# Autodesk Inventor assembly: Battery_pack
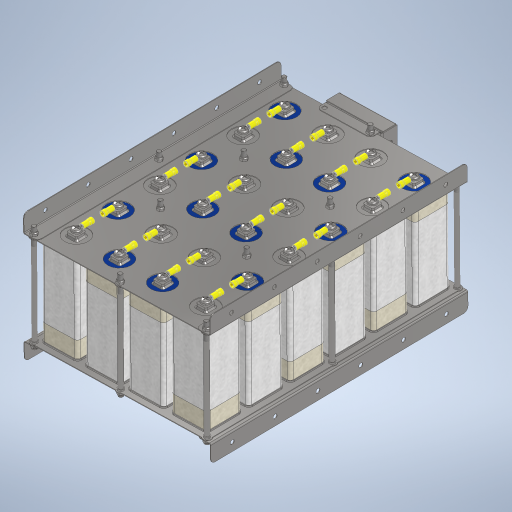
[picture p0: Inventor's stored thumbnail of the model, 512x512]
Saved by Autodesk Inventor 2023 (Build 270158000, 158)
## iProperties
Created: 2022-09-24
Part Number: Battery_pack
Document SubType Name: Assembly
Designer: dms01
Author: dms01
## Documents named in this file (16)
- D:\NEXT SPACE Lab\NaS battery\FINAL PROJECT\Battery_pack.iam
- D:\NEXT SPACE Lab\NaS battery\Frame.ipt
- D:\NEXT SPACE Lab\NaS battery\Square_cell.iam
- C:\Users\dms01\Documents\Inventor\Content Center Files\R2023\ru-RU\Stud GOST 22036-76\Шпилька M6-6g×140 ГОСТ 22036-76.ipt
- C:\Users\dms01\Documents\Inventor\Content Center Files\R2023\ru-RU\ANSI B18.16.3M(2)\ANSI B18.16.3M - Property Class 5 and 10 - Metric M5 x 0.8 Металлич..ipt
- C:\Users\dms01\Documents\Inventor\Content Center Files\R2023\ru-RU\Terminal Ring\#14 Terminal Ring 12 - 10 AWG.ipt
- C:\Users\dms01\Documents\Inventor\Content Center Files\R2023\ru-RU\KS B 1023  H (2)\KS B 1023 - A  M 6 x 8 - H(1).ipt
- C:\Users\dms01\Documents\Inventor\Content Center Files\R2023\ru-RU\D-Sub Female Crimp\D-Sub Female Crimp 9CKT.ipt
- D:\NEXT SPACE Lab\NaS battery\PCB_cover.ipt
- C:\Users\dms01\Documents\Inventor\Content Center Files\R2023\ru-RU\KS B 1023  H (2)\KS B 1023 - A  M 3 x 4 - H(1).ipt
- D:\NEXT SPACE Lab\NaS battery\Side_bar.ipt
- D:\NEXT SPACE Lab\NaS battery\Battery_pack\AIP\FEA\e3tpfgf5s.fins
- D:\NEXT SPACE Lab\NaS battery\Battery_pack\AIP\FEA\e3tpfgf6o.fsat
- D:\NEXT SPACE Lab\NaS battery\Battery_pack\AIP\FEA\e3tpfgf6o.ftes
- D:\NEXT SPACE Lab\NaS battery\Battery_pack\AIP\FEA\e3tpfgf6o.fwiz
- D:\NEXT SPACE Lab\NaS battery\Battery_pack\AIP\FEA\e3tpfghts.fmsh
## Components (168 placed, 10 different names)
1. Frame:1 — Жесткий:4, Вставка:1, Вставка:2, Вставка:3, Вставка:4, Вставка:5, Вставка:6, Вставка:7, Вставка:8, Вставка:9, Вставка:10, Вставка:11, Вставка:12, Вставка:14, Вставка:15, Вставка:16, Вставка:17, Вставка:19, Вставка:23, Жесткий:6, Жесткий:7, Жесткий:8, Жесткий:9, Жесткий:10, Жесткий:11, Жесткий:12, Жесткий:13, Жесткий:14, Жесткий:15, Жесткий:16, Симметрия:1, Жесткий:18, Жесткий:20, Жесткий:22, Жесткий:24, Жесткий:26, Жесткий:28, С поворотом:54, С поворотом:55
2. Frame:2 — Жесткий:5, Вставка:26, Вставка:28, Вставка:29, Вставка:30, Вставка:32, Симметрия:1, Жесткий:17, Жесткий:19, Жесткий:21, Жесткий:23, Жесткий:25, Жесткий:27, С поворотом:53, С поворотом:56, С поворотом:57
3. PCB_cover:1 — С поворотом:46, С поворотом:53, Вставка:104
4. D-Sub розетка, контакты под обжим D-Sub Female Crimp 9CKT:1 — С поворотом:46, Вставка:85, Вставка:86
5. Side_bar:1 — С поворотом:57, Вставка:92, Вставка:93, Вставка:94
6. Side_bar:2 — С поворотом:54, Вставка:101, Вставка:102, Вставка:103
7. Side_bar:3 — С поворотом:56, Вставка:95, Вставка:96, Вставка:97
8. Side_bar:4 — С поворотом:55, Вставка:98, Вставка:99, Вставка:100
9. Шпилька ГОСТ 22036-76 M6-6g×140:1 — Вставка:1
10. Шпилька ГОСТ 22036-76 M6-6g×140:2 — Вставка:2
11. Шпилька ГОСТ 22036-76 M6-6g×140:3 — Вставка:3
12. Шпилька ГОСТ 22036-76 M6-6g×140:4 — Вставка:4
13. Шпилька ГОСТ 22036-76 M6-6g×140:5 — Вставка:5
14. Шпилька ГОСТ 22036-76 M6-6g×140:6 — Вставка:6
15. Шпилька ГОСТ 22036-76 M6-6g×140:7 — Вставка:7
16. Шпилька ГОСТ 22036-76 M6-6g×140:8 — Вставка:8
17. Шпилька ГОСТ 22036-76 M6-6g×140:9 — Вставка:9
18. Шпилька ГОСТ 22036-76 M6-6g×140:10 — Вставка:10
19. Шпилька ГОСТ 22036-76 M6-6g×140:11 — Вставка:11
20. Шпилька ГОСТ 22036-76 M6-6g×140:12 — Вставка:12
21. Гайка шестигранная самоконтрящаяся - Сталь метрическая Property Class 5 and 10 - Metric M5 x 0.8 Металлич.:21 — Вставка:92
22. Гайка шестигранная самоконтрящаяся - Сталь метрическая Property Class 5 and 10 - Metric M5 x 0.8 Металлич.:22 — Вставка:93
23. Гайка шестигранная самоконтрящаяся - Сталь метрическая Property Class 5 and 10 - Metric M5 x 0.8 Металлич.:23 — Вставка:94
24. Гайка шестигранная самоконтрящаяся - Сталь метрическая Property Class 5 and 10 - Metric M5 x 0.8 Металлич.:24 — Вставка:95
25. Гайка шестигранная самоконтрящаяся - Сталь метрическая Property Class 5 and 10 - Metric M5 x 0.8 Металлич.:25 — Вставка:96
26. Гайка шестигранная самоконтрящаяся - Сталь метрическая Property Class 5 and 10 - Metric M5 x 0.8 Металлич.:26 — Вставка:97
27. Гайка шестигранная самоконтрящаяся - Сталь метрическая Property Class 5 and 10 - Metric M5 x 0.8 Металлич.:27 — Вставка:98
28. Гайка шестигранная самоконтрящаяся - Сталь метрическая Property Class 5 and 10 - Metric M5 x 0.8 Металлич.:28 — Вставка:99
29. Гайка шестигранная самоконтрящаяся - Сталь метрическая Property Class 5 and 10 - Metric M5 x 0.8 Металлич.:29 — Вставка:100
30. Гайка шестигранная самоконтрящаяся - Сталь метрическая Property Class 5 and 10 - Metric M5 x 0.8 Металлич.:30 — Вставка:101
31. Гайка шестигранная самоконтрящаяся - Сталь метрическая Property Class 5 and 10 - Metric M5 x 0.8 Металлич.:31 — Вставка:102
32. Гайка шестигранная самоконтрящаяся - Сталь метрическая Property Class 5 and 10 - Metric M5 x 0.8 Металлич.:32 — Вставка:103
33. Гайка шестигранная самоконтрящаяся - Сталь метрическая Property Class 5 and 10 - Metric M5 x 0.8 Металлич.:33 — Вставка:104
34. Гайка шестигранная самоконтрящаяся - Сталь метрическая Property Class 5 and 10 - Metric M5 x 0.8 Металлич.:2 — Вставка:14
35. Гайка шестигранная самоконтрящаяся - Сталь метрическая Property Class 5 and 10 - Metric M5 x 0.8 Металлич.:3 — Вставка:15
36. Гайка шестигранная самоконтрящаяся - Сталь метрическая Property Class 5 and 10 - Metric M5 x 0.8 Металлич.:4 — Вставка:16
37. Гайка шестигранная самоконтрящаяся - Сталь метрическая Property Class 5 and 10 - Metric M5 x 0.8 Металлич.:5 — Вставка:17
38. Гайка шестигранная самоконтрящаяся - Сталь метрическая Property Class 5 and 10 - Metric M5 x 0.8 Металлич.:7 — Вставка:19
39. Гайка шестигранная самоконтрящаяся - Сталь метрическая Property Class 5 and 10 - Metric M5 x 0.8 Металлич.:11 — Вставка:23
40. Гайка шестигранная самоконтрящаяся - Сталь метрическая Property Class 5 and 10 - Metric M5 x 0.8 Металлич.:14 — Вставка:26
41. Гайка шестигранная самоконтрящаяся - Сталь метрическая Property Class 5 and 10 - Metric M5 x 0.8 Металлич.:16 — Вставка:28
42. Гайка шестигранная самоконтрящаяся - Сталь метрическая Property Class 5 and 10 - Metric M5 x 0.8 Металлич.:17 — Вставка:29
43. Гайка шестигранная самоконтрящаяся - Сталь метрическая Property Class 5 and 10 - Metric M5 x 0.8 Металлич.:18 — Вставка:30
44. Гайка шестигранная самоконтрящаяся - Сталь метрическая Property Class 5 and 10 - Metric M5 x 0.8 Металлич.:20 — Вставка:32
45. Square_cell:8 [sub-assembly] — Жесткий:4, Жесткий:5, С поворотом:1, С поворотом:50
46. Square_cell:13 [sub-assembly] — Жесткий:10, С поворотом:10, С поворотом:11
47. Square_cell:12 [sub-assembly] — Жесткий:9, С поворотом:8, С поворотом:9
48. Square_cell:11 [sub-assembly] — Жесткий:8, С поворотом:6, С поворотом:7
49. Square_cell:10 [sub-assembly] — Жесткий:7, С поворотом:4, С поворотом:5
50. Square_cell:9 [sub-assembly] — Жесткий:6, С поворотом:2, С поворотом:3
51. Square_cell:19 [sub-assembly] — Жесткий:16, С поворотом:22, С поворотом:48
52. Square_cell:18 [sub-assembly] — Жесткий:15, С поворотом:20, С поворотом:21
53. Square_cell:17 [sub-assembly] — Жесткий:14, С поворотом:18, С поворотом:19
54. Square_cell:16 [sub-assembly] — Жесткий:13, С поворотом:16, С поворотом:17
55. Square_cell:15 [sub-assembly] — Жесткий:12, С поворотом:14, С поворотом:15
56. Square_cell:14 [sub-assembly] — Жесткий:11, С поворотом:12, С поворотом:13
57. Square_cell:20 [sub-assembly] — Жесткий:17, С поворотом:32, С поворотом:33
58. Square_cell:21 [sub-assembly] — Жесткий:18, С поворотом:30, С поворотом:31
59. Square_cell:22 [sub-assembly] — Жесткий:19, С поворотом:25, С поворотом:29
60. Square_cell:23 [sub-assembly] — Жесткий:20, С поворотом:26, С поворотом:28
61. Square_cell:24 [sub-assembly] — Жесткий:21, С поворотом:24, С поворотом:27
62. Square_cell:25 [sub-assembly] — Жесткий:22, С поворотом:23, С поворотом:47
63. Square_cell:26 [sub-assembly] — Жесткий:23, С поворотом:44, С поворотом:51
64. Square_cell:27 [sub-assembly] — Жесткий:24, С поворотом:40, С поворотом:43
65. Square_cell:28 [sub-assembly] — Жесткий:25, С поворотом:39, С поворотом:42
66. Square_cell:29 [sub-assembly] — Жесткий:26, С поворотом:38, С поворотом:41
67. Square_cell:30 [sub-assembly] — Жесткий:27, С поворотом:36, С поворотом:37
68. Square_cell:31 [sub-assembly] — Жесткий:28, С поворотом:34, С поворотом:35
69. Кольцевой зажим #14 Terminal Ring 12 - 10 AWG:45 — С поворотом:47, Вставка:89
70. Кольцевой зажим #14 Terminal Ring 12 - 10 AWG:46 — С поворотом:48, С поворотом:49
71. Кольцевой зажим #14 Terminal Ring 12 - 10 AWG:47 — С поворотом:49, Вставка:90
72. Кольцевой зажим #14 Terminal Ring 12 - 10 AWG:48 — С поворотом:50, С поворотом:52
73. Кольцевой зажим #14 Terminal Ring 12 - 10 AWG:49 — С поворотом:51, Вставка:88
74. Кольцевой зажим #14 Terminal Ring 12 - 10 AWG:50 — С поворотом:52, Вставка:91
75. Кольцевой зажим #14 Terminal Ring 12 - 10 AWG:1 — С поворотом:1, Вставка:57
76. Кольцевой зажим #14 Terminal Ring 12 - 10 AWG:2 — С поворотом:2, Вставка:56
77. Кольцевой зажим #14 Terminal Ring 12 - 10 AWG:3 — С поворотом:10, Вставка:48
78. Кольцевой зажим #14 Terminal Ring 12 - 10 AWG:4 — С поворотом:9, Вставка:46
79. Кольцевой зажим #14 Terminal Ring 12 - 10 AWG:5 — С поворотом:7, Вставка:69
80. Кольцевой зажим #14 Terminal Ring 12 - 10 AWG:6 — С поворотом:8, Вставка:68
81. Кольцевой зажим #14 Terminal Ring 12 - 10 AWG:7 — С поворотом:5, Вставка:49
82. Кольцевой зажим #14 Terminal Ring 12 - 10 AWG:8 — С поворотом:6, Вставка:47
83. Кольцевой зажим #14 Terminal Ring 12 - 10 AWG:9 — С поворотом:3, Вставка:80
84. Кольцевой зажим #14 Terminal Ring 12 - 10 AWG:10 — С поворотом:4, Вставка:73
85. Кольцевой зажим #14 Terminal Ring 12 - 10 AWG:11 — С поворотом:20, Вставка:79
86. Кольцевой зажим #14 Terminal Ring 12 - 10 AWG:12 — С поворотом:19, Вставка:74
87. Кольцевой зажим #14 Terminal Ring 12 - 10 AWG:13 — С поворотом:18, Вставка:50
88. Кольцевой зажим #14 Terminal Ring 12 - 10 AWG:14 — С поворотом:17, Вставка:45
89. Кольцевой зажим #14 Terminal Ring 12 - 10 AWG:15 — С поворотом:16, Вставка:70
90. Кольцевой зажим #14 Terminal Ring 12 - 10 AWG:16 — С поворотом:15, Вставка:67
91. Кольцевой зажим #14 Terminal Ring 12 - 10 AWG:17 — С поворотом:14, Вставка:42
92. Кольцевой зажим #14 Terminal Ring 12 - 10 AWG:18 — С поворотом:13, Вставка:39
93. Кольцевой зажим #14 Terminal Ring 12 - 10 AWG:19 — С поворотом:12, Вставка:62
94. Кольцевой зажим #14 Terminal Ring 12 - 10 AWG:20 — С поворотом:11, Вставка:61
95. Кольцевой зажим #14 Terminal Ring 12 - 10 AWG:21 — С поворотом:22, Вставка:58
96. Кольцевой зажим #14 Terminal Ring 12 - 10 AWG:22 — С поворотом:21, Вставка:55
97. Кольцевой зажим #14 Terminal Ring 12 - 10 AWG:23 — С поворотом:23, Вставка:59
98. Кольцевой зажим #14 Terminal Ring 12 - 10 AWG:24 — С поворотом:25, Вставка:43
99. Кольцевой зажим #14 Terminal Ring 12 - 10 AWG:25 — С поворотом:27, Вставка:78
100. Кольцевой зажим #14 Terminal Ring 12 - 10 AWG:26 — С поворотом:29, Вставка:71
101. Кольцевой зажим #14 Terminal Ring 12 - 10 AWG:27 — С поворотом:40, Вставка:77
102. Кольцевой зажим #14 Terminal Ring 12 - 10 AWG:28 — С поворотом:38, Вставка:72
103. Кольцевой зажим #14 Terminal Ring 12 - 10 AWG:29 — С поворотом:37, Вставка:65
104. Кольцевой зажим #14 Terminal Ring 12 - 10 AWG:30 — С поворотом:35, Вставка:37
105. Кольцевой зажим #14 Terminal Ring 12 - 10 AWG:31 — С поворотом:33, Вставка:63
106. Кольцевой зажим #14 Terminal Ring 12 - 10 AWG:32 — С поворотом:32, Вставка:38
107. Кольцевой зажим #14 Terminal Ring 12 - 10 AWG:33 — С поворотом:31, Вставка:40
108. Кольцевой зажим #14 Terminal Ring 12 - 10 AWG:34 — С поворотом:34, Вставка:64
109. Кольцевой зажим #14 Terminal Ring 12 - 10 AWG:35 — С поворотом:36, Вставка:41
110. Кольцевой зажим #14 Terminal Ring 12 - 10 AWG:36 — С поворотом:39, Вставка:76
111. Кольцевой зажим #14 Terminal Ring 12 - 10 AWG:37 — С поворотом:41, Вставка:44
112. Кольцевой зажим #14 Terminal Ring 12 - 10 AWG:38 — С поворотом:42, Вставка:52
113. Кольцевой зажим #14 Terminal Ring 12 - 10 AWG:39 — С поворотом:30, Вставка:66
114. Кольцевой зажим #14 Terminal Ring 12 - 10 AWG:40 — С поворотом:28, Вставка:75
115. Кольцевой зажим #14 Terminal Ring 12 - 10 AWG:41 — С поворотом:26, Вставка:51
116. Кольцевой зажим #14 Terminal Ring 12 - 10 AWG:42 — С поворотом:24, Вставка:54
117. Кольцевой зажим #14 Terminal Ring 12 - 10 AWG:43 — С поворотом:43, Вставка:53
118. Кольцевой зажим #14 Terminal Ring 12 - 10 AWG:44 — С поворотом:44, Вставка:60
119. KS B 1023 H - метрическая A  M 6 x 8 - H:45 — Вставка:88
120. KS B 1023 H - метрическая A  M 6 x 8 - H:46 — Вставка:89
121. KS B 1023 H - метрическая A  M 6 x 8 - H:47 — Вставка:90
122. KS B 1023 H - метрическая A  M 6 x 8 - H:48 — Вставка:91
123. KS B 1023 H - метрическая A  M 3 x 4 - H:1 — Вставка:85
124. KS B 1023 H - метрическая A  M 3 x 4 - H:2 — Вставка:86
125. KS B 1023 H - метрическая A  M 6 x 8 - H:1 — Вставка:37
126. KS B 1023 H - метрическая A  M 6 x 8 - H:2 — Вставка:38
127. KS B 1023 H - метрическая A  M 6 x 8 - H:3 — Вставка:39
128. KS B 1023 H - метрическая A  M 6 x 8 - H:4 — Вставка:40
129. KS B 1023 H - метрическая A  M 6 x 8 - H:5 — Вставка:41
130. KS B 1023 H - метрическая A  M 6 x 8 - H:6 — Вставка:42
131. KS B 1023 H - метрическая A  M 6 x 8 - H:7 — Вставка:43
132. KS B 1023 H - метрическая A  M 6 x 8 - H:8 — Вставка:44
133. KS B 1023 H - метрическая A  M 6 x 8 - H:9 — Вставка:45
134. KS B 1023 H - метрическая A  M 6 x 8 - H:10 — Вставка:46
135. KS B 1023 H - метрическая A  M 6 x 8 - H:11 — Вставка:47
136. KS B 1023 H - метрическая A  M 6 x 8 - H:12 — Вставка:48
137. KS B 1023 H - метрическая A  M 6 x 8 - H:13 — Вставка:49
138. KS B 1023 H - метрическая A  M 6 x 8 - H:14 — Вставка:50
139. KS B 1023 H - метрическая A  M 6 x 8 - H:15 — Вставка:51
140. KS B 1023 H - метрическая A  M 6 x 8 - H:16 — Вставка:52
141. KS B 1023 H - метрическая A  M 6 x 8 - H:17 — Вставка:53
142. KS B 1023 H - метрическая A  M 6 x 8 - H:18 — Вставка:54
143. KS B 1023 H - метрическая A  M 6 x 8 - H:19 — Вставка:55
144. KS B 1023 H - метрическая A  M 6 x 8 - H:20 — Вставка:56
145. KS B 1023 H - метрическая A  M 6 x 8 - H:21 — Вставка:57
146. KS B 1023 H - метрическая A  M 6 x 8 - H:22 — Вставка:58
147. KS B 1023 H - метрическая A  M 6 x 8 - H:23 — Вставка:59
148. KS B 1023 H - метрическая A  M 6 x 8 - H:24 — Вставка:60
149. KS B 1023 H - метрическая A  M 6 x 8 - H:25 — Вставка:61
150. KS B 1023 H - метрическая A  M 6 x 8 - H:26 — Вставка:62
151. KS B 1023 H - метрическая A  M 6 x 8 - H:27 — Вставка:63
152. KS B 1023 H - метрическая A  M 6 x 8 - H:28 — Вставка:64
153. KS B 1023 H - метрическая A  M 6 x 8 - H:29 — Вставка:65
154. KS B 1023 H - метрическая A  M 6 x 8 - H:30 — Вставка:66
155. KS B 1023 H - метрическая A  M 6 x 8 - H:31 — Вставка:67
156. KS B 1023 H - метрическая A  M 6 x 8 - H:32 — Вставка:68
157. KS B 1023 H - метрическая A  M 6 x 8 - H:33 — Вставка:69
158. KS B 1023 H - метрическая A  M 6 x 8 - H:34 — Вставка:70
159. KS B 1023 H - метрическая A  M 6 x 8 - H:35 — Вставка:71
160. KS B 1023 H - метрическая A  M 6 x 8 - H:36 — Вставка:72
161. KS B 1023 H - метрическая A  M 6 x 8 - H:37 — Вставка:73
162. KS B 1023 H - метрическая A  M 6 x 8 - H:38 — Вставка:74
163. KS B 1023 H - метрическая A  M 6 x 8 - H:39 — Вставка:75
164. KS B 1023 H - метрическая A  M 6 x 8 - H:40 — Вставка:76
165. KS B 1023 H - метрическая A  M 6 x 8 - H:41 — Вставка:77
166. KS B 1023 H - метрическая A  M 6 x 8 - H:42 — Вставка:78
167. KS B 1023 H - метрическая A  M 6 x 8 - H:43 — Вставка:79
168. KS B 1023 H - метрическая A  M 6 x 8 - H:44 — Вставка:80
## Relationships (168: Insert 86, RevoluteJoint 56, WeldJoint 25, Symmetry 1)
- Жесткий:4 [WeldJoint]: Frame:1 ↔ Square_cell:8
- Жесткий:5 [WeldJoint]: Frame:2 ↔ Square_cell:8
- Вставка:1 [Insert]: Frame:1 ↔ Шпилька ГОСТ 22036-76 M6-6g×140:1
- Вставка:2 [Insert]: Frame:1 ↔ Шпилька ГОСТ 22036-76 M6-6g×140:2
- Вставка:3 [Insert]: Frame:1 ↔ Шпилька ГОСТ 22036-76 M6-6g×140:3
- Вставка:4 [Insert]: Frame:1 ↔ Шпилька ГОСТ 22036-76 M6-6g×140:4
- Вставка:5 [Insert]: Frame:1 ↔ Шпилька ГОСТ 22036-76 M6-6g×140:5
- Вставка:6 [Insert]: Frame:1 ↔ Шпилька ГОСТ 22036-76 M6-6g×140:6
- Вставка:7 [Insert]: Frame:1 ↔ Шпилька ГОСТ 22036-76 M6-6g×140:7
- Вставка:8 [Insert]: Frame:1 ↔ Шпилька ГОСТ 22036-76 M6-6g×140:8
- Вставка:9 [Insert]: Frame:1 ↔ Шпилька ГОСТ 22036-76 M6-6g×140:9
- Вставка:10 [Insert]: Frame:1 ↔ Шпилька ГОСТ 22036-76 M6-6g×140:10
- Вставка:11 [Insert]: Frame:1 ↔ Шпилька ГОСТ 22036-76 M6-6g×140:11
- Вставка:12 [Insert]: Frame:1 ↔ Шпилька ГОСТ 22036-76 M6-6g×140:12
- Вставка:14 [Insert]: Frame:1 ↔ Гайка шестигранная самоконтрящаяся - Сталь метрическая Property Class 5 and 10 - Metric M5 x 0.8 Металлич.:2
- Вставка:15 [Insert]: Frame:1 ↔ Гайка шестигранная самоконтрящаяся - Сталь метрическая Property Class 5 and 10 - Metric M5 x 0.8 Металлич.:3
- Вставка:16 [Insert]: Frame:1 ↔ Гайка шестигранная самоконтрящаяся - Сталь метрическая Property Class 5 and 10 - Metric M5 x 0.8 Металлич.:4
- Вставка:17 [Insert]: Frame:1 ↔ Гайка шестигранная самоконтрящаяся - Сталь метрическая Property Class 5 and 10 - Metric M5 x 0.8 Металлич.:5
- Вставка:19 [Insert]: Frame:1 ↔ Гайка шестигранная самоконтрящаяся - Сталь метрическая Property Class 5 and 10 - Metric M5 x 0.8 Металлич.:7
- Вставка:23 [Insert]: Frame:1 ↔ Гайка шестигранная самоконтрящаяся - Сталь метрическая Property Class 5 and 10 - Metric M5 x 0.8 Металлич.:11
- Вставка:26 [Insert]: Frame:2 ↔ Гайка шестигранная самоконтрящаяся - Сталь метрическая Property Class 5 and 10 - Metric M5 x 0.8 Металлич.:14
- Вставка:28 [Insert]: Frame:2 ↔ Гайка шестигранная самоконтрящаяся - Сталь метрическая Property Class 5 and 10 - Metric M5 x 0.8 Металлич.:16
- Вставка:29 [Insert]: Frame:2 ↔ Гайка шестигранная самоконтрящаяся - Сталь метрическая Property Class 5 and 10 - Metric M5 x 0.8 Металлич.:17
- Вставка:30 [Insert]: Frame:2 ↔ Гайка шестигранная самоконтрящаяся - Сталь метрическая Property Class 5 and 10 - Metric M5 x 0.8 Металлич.:18
- Вставка:32 [Insert]: Frame:2 ↔ Гайка шестигранная самоконтрящаяся - Сталь метрическая Property Class 5 and 10 - Metric M5 x 0.8 Металлич.:20
- Жесткий:6 [WeldJoint]: Frame:1 ↔ Square_cell:9
- Жесткий:7 [WeldJoint]: Frame:1 ↔ Square_cell:10
- Жесткий:8 [WeldJoint]: Frame:1 ↔ Square_cell:11
- Жесткий:9 [WeldJoint]: Frame:1 ↔ Square_cell:12
- Жесткий:10 [WeldJoint]: Frame:1 ↔ Square_cell:13
- Жесткий:11 [WeldJoint]: Frame:1 ↔ Square_cell:14
- Жесткий:12 [WeldJoint]: Frame:1 ↔ Square_cell:15
- Жесткий:13 [WeldJoint]: Frame:1 ↔ Square_cell:16
- Жесткий:14 [WeldJoint]: Frame:1 ↔ Square_cell:17
- Жесткий:15 [WeldJoint]: Frame:1 ↔ Square_cell:18
- Жесткий:16 [WeldJoint]: Frame:1 ↔ Square_cell:19
- Симметрия:1 [Symmetry]: Frame:1 ↔ Frame:2
- Жесткий:17 [WeldJoint]: Frame:2 ↔ Square_cell:20
- Жесткий:18 [WeldJoint]: Frame:1 ↔ Square_cell:21
- Жесткий:19 [WeldJoint]: Frame:2 ↔ Square_cell:22
- Жесткий:20 [WeldJoint]: Frame:1 ↔ Square_cell:23
- Жесткий:21 [WeldJoint]: Frame:2 ↔ Square_cell:24
- Жесткий:22 [WeldJoint]: Frame:1 ↔ Square_cell:25
- Жесткий:23 [WeldJoint]: Frame:2 ↔ Square_cell:26
- Жесткий:24 [WeldJoint]: Frame:1 ↔ Square_cell:27
- Жесткий:25 [WeldJoint]: Frame:2 ↔ Square_cell:28
- Жесткий:26 [WeldJoint]: Frame:1 ↔ Square_cell:29
- Жесткий:27 [WeldJoint]: Frame:2 ↔ Square_cell:30
- Жесткий:28 [WeldJoint]: Frame:1 ↔ Square_cell:31
- С поворотом:1 [RevoluteJoint]: Square_cell:8 ↔ Кольцевой зажим #14 Terminal Ring 12 - 10 AWG:1
- С поворотом:2 [RevoluteJoint]: Square_cell:9 ↔ Кольцевой зажим #14 Terminal Ring 12 - 10 AWG:2
- С поворотом:3 [RevoluteJoint]: Square_cell:9 ↔ Кольцевой зажим #14 Terminal Ring 12 - 10 AWG:9
- С поворотом:4 [RevoluteJoint]: Square_cell:10 ↔ Кольцевой зажим #14 Terminal Ring 12 - 10 AWG:10
- С поворотом:5 [RevoluteJoint]: Square_cell:10 ↔ Кольцевой зажим #14 Terminal Ring 12 - 10 AWG:7
- С поворотом:6 [RevoluteJoint]: Square_cell:11 ↔ Кольцевой зажим #14 Terminal Ring 12 - 10 AWG:8
- С поворотом:7 [RevoluteJoint]: Square_cell:11 ↔ Кольцевой зажим #14 Terminal Ring 12 - 10 AWG:5
- С поворотом:8 [RevoluteJoint]: Square_cell:12 ↔ Кольцевой зажим #14 Terminal Ring 12 - 10 AWG:6
- С поворотом:9 [RevoluteJoint]: Square_cell:12 ↔ Кольцевой зажим #14 Terminal Ring 12 - 10 AWG:4
- С поворотом:10 [RevoluteJoint]: Square_cell:13 ↔ Кольцевой зажим #14 Terminal Ring 12 - 10 AWG:3
- С поворотом:11 [RevoluteJoint]: Square_cell:13 ↔ Кольцевой зажим #14 Terminal Ring 12 - 10 AWG:20
- С поворотом:12 [RevoluteJoint]: Square_cell:14 ↔ Кольцевой зажим #14 Terminal Ring 12 - 10 AWG:19
- С поворотом:13 [RevoluteJoint]: Square_cell:14 ↔ Кольцевой зажим #14 Terminal Ring 12 - 10 AWG:18
- С поворотом:14 [RevoluteJoint]: Square_cell:15 ↔ Кольцевой зажим #14 Terminal Ring 12 - 10 AWG:17
- С поворотом:15 [RevoluteJoint]: Square_cell:15 ↔ Кольцевой зажим #14 Terminal Ring 12 - 10 AWG:16
- С поворотом:16 [RevoluteJoint]: Square_cell:16 ↔ Кольцевой зажим #14 Terminal Ring 12 - 10 AWG:15
- С поворотом:17 [RevoluteJoint]: Square_cell:16 ↔ Кольцевой зажим #14 Terminal Ring 12 - 10 AWG:14
- С поворотом:18 [RevoluteJoint]: Square_cell:17 ↔ Кольцевой зажим #14 Terminal Ring 12 - 10 AWG:13
- С поворотом:19 [RevoluteJoint]: Square_cell:17 ↔ Кольцевой зажим #14 Terminal Ring 12 - 10 AWG:12
- С поворотом:20 [RevoluteJoint]: Square_cell:18 ↔ Кольцевой зажим #14 Terminal Ring 12 - 10 AWG:11
- С поворотом:21 [RevoluteJoint]: Square_cell:18 ↔ Кольцевой зажим #14 Terminal Ring 12 - 10 AWG:22
- С поворотом:22 [RevoluteJoint]: Square_cell:19 ↔ Кольцевой зажим #14 Terminal Ring 12 - 10 AWG:21
- С поворотом:23 [RevoluteJoint]: Square_cell:25 ↔ Кольцевой зажим #14 Terminal Ring 12 - 10 AWG:23
- С поворотом:24 [RevoluteJoint]: Square_cell:24 ↔ Кольцевой зажим #14 Terminal Ring 12 - 10 AWG:42
- С поворотом:25 [RevoluteJoint]: Square_cell:22 ↔ Кольцевой зажим #14 Terminal Ring 12 - 10 AWG:24
- С поворотом:26 [RevoluteJoint]: Square_cell:23 ↔ Кольцевой зажим #14 Terminal Ring 12 - 10 AWG:41
- С поворотом:27 [RevoluteJoint]: Square_cell:24 ↔ Кольцевой зажим #14 Terminal Ring 12 - 10 AWG:25
- С поворотом:28 [RevoluteJoint]: Square_cell:23 ↔ Кольцевой зажим #14 Terminal Ring 12 - 10 AWG:40
- С поворотом:29 [RevoluteJoint]: Square_cell:22 ↔ Кольцевой зажим #14 Terminal Ring 12 - 10 AWG:26
- С поворотом:30 [RevoluteJoint]: Square_cell:21 ↔ Кольцевой зажим #14 Terminal Ring 12 - 10 AWG:39
- С поворотом:31 [RevoluteJoint]: Square_cell:21 ↔ Кольцевой зажим #14 Terminal Ring 12 - 10 AWG:33
- С поворотом:32 [RevoluteJoint]: Square_cell:20 ↔ Кольцевой зажим #14 Terminal Ring 12 - 10 AWG:32
- С поворотом:33 [RevoluteJoint]: Square_cell:20 ↔ Кольцевой зажим #14 Terminal Ring 12 - 10 AWG:31
- С поворотом:34 [RevoluteJoint]: Square_cell:31 ↔ Кольцевой зажим #14 Terminal Ring 12 - 10 AWG:34
- С поворотом:35 [RevoluteJoint]: Square_cell:31 ↔ Кольцевой зажим #14 Terminal Ring 12 - 10 AWG:30
- С поворотом:36 [RevoluteJoint]: Square_cell:30 ↔ Кольцевой зажим #14 Terminal Ring 12 - 10 AWG:35
- С поворотом:37 [RevoluteJoint]: Square_cell:30 ↔ Кольцевой зажим #14 Terminal Ring 12 - 10 AWG:29
- С поворотом:38 [RevoluteJoint]: Square_cell:29 ↔ Кольцевой зажим #14 Terminal Ring 12 - 10 AWG:28
- С поворотом:39 [RevoluteJoint]: Square_cell:28 ↔ Кольцевой зажим #14 Terminal Ring 12 - 10 AWG:36
- С поворотом:40 [RevoluteJoint]: Square_cell:27 ↔ Кольцевой зажим #14 Terminal Ring 12 - 10 AWG:27
- С поворотом:41 [RevoluteJoint]: Square_cell:29 ↔ Кольцевой зажим #14 Terminal Ring 12 - 10 AWG:37
- С поворотом:42 [RevoluteJoint]: Square_cell:28 ↔ Кольцевой зажим #14 Terminal Ring 12 - 10 AWG:38
- С поворотом:43 [RevoluteJoint]: Square_cell:27 ↔ Кольцевой зажим #14 Terminal Ring 12 - 10 AWG:43
- С поворотом:44 [RevoluteJoint]: Square_cell:26 ↔ Кольцевой зажим #14 Terminal Ring 12 - 10 AWG:44
- Вставка:37 [Insert]: Кольцевой зажим #14 Terminal Ring 12 - 10 AWG:30 ↔ KS B 1023 H - метрическая A  M 6 x 8 - H:1
- Вставка:38 [Insert]: Кольцевой зажим #14 Terminal Ring 12 - 10 AWG:32 ↔ KS B 1023 H - метрическая A  M 6 x 8 - H:2
- Вставка:39 [Insert]: Кольцевой зажим #14 Terminal Ring 12 - 10 AWG:18 ↔ KS B 1023 H - метрическая A  M 6 x 8 - H:3
- Вставка:40 [Insert]: Кольцевой зажим #14 Terminal Ring 12 - 10 AWG:33 ↔ KS B 1023 H - метрическая A  M 6 x 8 - H:4
- Вставка:41 [Insert]: Кольцевой зажим #14 Terminal Ring 12 - 10 AWG:35 ↔ KS B 1023 H - метрическая A  M 6 x 8 - H:5
- Вставка:42 [Insert]: Кольцевой зажим #14 Terminal Ring 12 - 10 AWG:17 ↔ KS B 1023 H - метрическая A  M 6 x 8 - H:6
- Вставка:43 [Insert]: Кольцевой зажим #14 Terminal Ring 12 - 10 AWG:24 ↔ KS B 1023 H - метрическая A  M 6 x 8 - H:7
- Вставка:44 [Insert]: Кольцевой зажим #14 Terminal Ring 12 - 10 AWG:37 ↔ KS B 1023 H - метрическая A  M 6 x 8 - H:8
- Вставка:45 [Insert]: Кольцевой зажим #14 Terminal Ring 12 - 10 AWG:14 ↔ KS B 1023 H - метрическая A  M 6 x 8 - H:9
- Вставка:46 [Insert]: Кольцевой зажим #14 Terminal Ring 12 - 10 AWG:4 ↔ KS B 1023 H - метрическая A  M 6 x 8 - H:10
- Вставка:47 [Insert]: Кольцевой зажим #14 Terminal Ring 12 - 10 AWG:8 ↔ KS B 1023 H - метрическая A  M 6 x 8 - H:11
- Вставка:48 [Insert]: Кольцевой зажим #14 Terminal Ring 12 - 10 AWG:3 ↔ KS B 1023 H - метрическая A  M 6 x 8 - H:12
- Вставка:49 [Insert]: Кольцевой зажим #14 Terminal Ring 12 - 10 AWG:7 ↔ KS B 1023 H - метрическая A  M 6 x 8 - H:13
- Вставка:50 [Insert]: Кольцевой зажим #14 Terminal Ring 12 - 10 AWG:13 ↔ KS B 1023 H - метрическая A  M 6 x 8 - H:14
- Вставка:51 [Insert]: Кольцевой зажим #14 Terminal Ring 12 - 10 AWG:41 ↔ KS B 1023 H - метрическая A  M 6 x 8 - H:15
- Вставка:52 [Insert]: Кольцевой зажим #14 Terminal Ring 12 - 10 AWG:38 ↔ KS B 1023 H - метрическая A  M 6 x 8 - H:16
- Вставка:53 [Insert]: Кольцевой зажим #14 Terminal Ring 12 - 10 AWG:43 ↔ KS B 1023 H - метрическая A  M 6 x 8 - H:17
- Вставка:54 [Insert]: Кольцевой зажим #14 Terminal Ring 12 - 10 AWG:42 ↔ KS B 1023 H - метрическая A  M 6 x 8 - H:18
- Вставка:55 [Insert]: Кольцевой зажим #14 Terminal Ring 12 - 10 AWG:22 ↔ KS B 1023 H - метрическая A  M 6 x 8 - H:19
- Вставка:56 [Insert]: Кольцевой зажим #14 Terminal Ring 12 - 10 AWG:2 ↔ KS B 1023 H - метрическая A  M 6 x 8 - H:20
- Вставка:57 [Insert]: Кольцевой зажим #14 Terminal Ring 12 - 10 AWG:1 ↔ KS B 1023 H - метрическая A  M 6 x 8 - H:21
- Вставка:58 [Insert]: Кольцевой зажим #14 Terminal Ring 12 - 10 AWG:21 ↔ KS B 1023 H - метрическая A  M 6 x 8 - H:22
- Вставка:59 [Insert]: Кольцевой зажим #14 Terminal Ring 12 - 10 AWG:23 ↔ KS B 1023 H - метрическая A  M 6 x 8 - H:23
- Вставка:60 [Insert]: Кольцевой зажим #14 Terminal Ring 12 - 10 AWG:44 ↔ KS B 1023 H - метрическая A  M 6 x 8 - H:24
- Вставка:61 [Insert]: Кольцевой зажим #14 Terminal Ring 12 - 10 AWG:20 ↔ KS B 1023 H - метрическая A  M 6 x 8 - H:25
- Вставка:62 [Insert]: Кольцевой зажим #14 Terminal Ring 12 - 10 AWG:19 ↔ KS B 1023 H - метрическая A  M 6 x 8 - H:26
- Вставка:63 [Insert]: Кольцевой зажим #14 Terminal Ring 12 - 10 AWG:31 ↔ KS B 1023 H - метрическая A  M 6 x 8 - H:27
- Вставка:64 [Insert]: Кольцевой зажим #14 Terminal Ring 12 - 10 AWG:34 ↔ KS B 1023 H - метрическая A  M 6 x 8 - H:28
- Вставка:65 [Insert]: Кольцевой зажим #14 Terminal Ring 12 - 10 AWG:29 ↔ KS B 1023 H - метрическая A  M 6 x 8 - H:29
- Вставка:66 [Insert]: Кольцевой зажим #14 Terminal Ring 12 - 10 AWG:39 ↔ KS B 1023 H - метрическая A  M 6 x 8 - H:30
- Вставка:67 [Insert]: Кольцевой зажим #14 Terminal Ring 12 - 10 AWG:16 ↔ KS B 1023 H - метрическая A  M 6 x 8 - H:31
- Вставка:68 [Insert]: Кольцевой зажим #14 Terminal Ring 12 - 10 AWG:6 ↔ KS B 1023 H - метрическая A  M 6 x 8 - H:32
- Вставка:69 [Insert]: Кольцевой зажим #14 Terminal Ring 12 - 10 AWG:5 ↔ KS B 1023 H - метрическая A  M 6 x 8 - H:33
- Вставка:70 [Insert]: Кольцевой зажим #14 Terminal Ring 12 - 10 AWG:15 ↔ KS B 1023 H - метрическая A  M 6 x 8 - H:34
- Вставка:71 [Insert]: Кольцевой зажим #14 Terminal Ring 12 - 10 AWG:26 ↔ KS B 1023 H - метрическая A  M 6 x 8 - H:35
- Вставка:72 [Insert]: Кольцевой зажим #14 Terminal Ring 12 - 10 AWG:28 ↔ KS B 1023 H - метрическая A  M 6 x 8 - H:36
- Вставка:73 [Insert]: Кольцевой зажим #14 Terminal Ring 12 - 10 AWG:10 ↔ KS B 1023 H - метрическая A  M 6 x 8 - H:37
- Вставка:74 [Insert]: Кольцевой зажим #14 Terminal Ring 12 - 10 AWG:12 ↔ KS B 1023 H - метрическая A  M 6 x 8 - H:38
- Вставка:75 [Insert]: Кольцевой зажим #14 Terminal Ring 12 - 10 AWG:40 ↔ KS B 1023 H - метрическая A  M 6 x 8 - H:39
- Вставка:76 [Insert]: Кольцевой зажим #14 Terminal Ring 12 - 10 AWG:36 ↔ KS B 1023 H - метрическая A  M 6 x 8 - H:40
- Вставка:77 [Insert]: Кольцевой зажим #14 Terminal Ring 12 - 10 AWG:27 ↔ KS B 1023 H - метрическая A  M 6 x 8 - H:41
- Вставка:78 [Insert]: Кольцевой зажим #14 Terminal Ring 12 - 10 AWG:25 ↔ KS B 1023 H - метрическая A  M 6 x 8 - H:42
- Вставка:79 [Insert]: Кольцевой зажим #14 Terminal Ring 12 - 10 AWG:11 ↔ KS B 1023 H - метрическая A  M 6 x 8 - H:43
- Вставка:80 [Insert]: Кольцевой зажим #14 Terminal Ring 12 - 10 AWG:9 ↔ KS B 1023 H - метрическая A  M 6 x 8 - H:44
- С поворотом:46 [RevoluteJoint]: PCB_cover:1 ↔ D-Sub розетка, контакты под обжим D-Sub Female Crimp 9CKT:1
- Вставка:85 [Insert]: D-Sub розетка, контакты под обжим D-Sub Female Crimp 9CKT:1 ↔ KS B 1023 H - метрическая A  M 3 x 4 - H:1
- Вставка:86 [Insert]: D-Sub розетка, контакты под обжим D-Sub Female Crimp 9CKT:1 ↔ KS B 1023 H - метрическая A  M 3 x 4 - H:2
- С поворотом:47 [RevoluteJoint]: Square_cell:25 ↔ Кольцевой зажим #14 Terminal Ring 12 - 10 AWG:45
- С поворотом:48 [RevoluteJoint]: Square_cell:19 ↔ Кольцевой зажим #14 Terminal Ring 12 - 10 AWG:46
- С поворотом:49 [RevoluteJoint]: Кольцевой зажим #14 Terminal Ring 12 - 10 AWG:46 ↔ Кольцевой зажим #14 Terminal Ring 12 - 10 AWG:47
- С поворотом:50 [RevoluteJoint]: Square_cell:8 ↔ Кольцевой зажим #14 Terminal Ring 12 - 10 AWG:48
- С поворотом:51 [RevoluteJoint]: Square_cell:26 ↔ Кольцевой зажим #14 Terminal Ring 12 - 10 AWG:49
- С поворотом:52 [RevoluteJoint]: Кольцевой зажим #14 Terminal Ring 12 - 10 AWG:48 ↔ Кольцевой зажим #14 Terminal Ring 12 - 10 AWG:50
- Вставка:88 [Insert]: Кольцевой зажим #14 Terminal Ring 12 - 10 AWG:49 ↔ KS B 1023 H - метрическая A  M 6 x 8 - H:45
- Вставка:89 [Insert]: Кольцевой зажим #14 Terminal Ring 12 - 10 AWG:45 ↔ KS B 1023 H - метрическая A  M 6 x 8 - H:46
- Вставка:90 [Insert]: Кольцевой зажим #14 Terminal Ring 12 - 10 AWG:47 ↔ KS B 1023 H - метрическая A  M 6 x 8 - H:47
- Вставка:91 [Insert]: Кольцевой зажим #14 Terminal Ring 12 - 10 AWG:50 ↔ KS B 1023 H - метрическая A  M 6 x 8 - H:48
- С поворотом:53 [RevoluteJoint]: Frame:2 ↔ PCB_cover:1
- С поворотом:54 [RevoluteJoint]: Frame:1 ↔ Side_bar:2
- С поворотом:55 [RevoluteJoint]: Frame:1 ↔ Side_bar:4
- С поворотом:56 [RevoluteJoint]: Frame:2 ↔ Side_bar:3
- С поворотом:57 [RevoluteJoint]: Frame:2 ↔ Side_bar:1
- Вставка:92 [Insert]: Side_bar:1 ↔ Гайка шестигранная самоконтрящаяся - Сталь метрическая Property Class 5 and 10 - Metric M5 x 0.8 Металлич.:21
- Вставка:93 [Insert]: Side_bar:1 ↔ Гайка шестигранная самоконтрящаяся - Сталь метрическая Property Class 5 and 10 - Metric M5 x 0.8 Металлич.:22
- Вставка:94 [Insert]: Side_bar:1 ↔ Гайка шестигранная самоконтрящаяся - Сталь метрическая Property Class 5 and 10 - Metric M5 x 0.8 Металлич.:23
- Вставка:95 [Insert]: Side_bar:3 ↔ Гайка шестигранная самоконтрящаяся - Сталь метрическая Property Class 5 and 10 - Metric M5 x 0.8 Металлич.:24
- Вставка:96 [Insert]: Side_bar:3 ↔ Гайка шестигранная самоконтрящаяся - Сталь метрическая Property Class 5 and 10 - Metric M5 x 0.8 Металлич.:25
- Вставка:97 [Insert]: Side_bar:3 ↔ Гайка шестигранная самоконтрящаяся - Сталь метрическая Property Class 5 and 10 - Metric M5 x 0.8 Металлич.:26
- Вставка:98 [Insert]: Side_bar:4 ↔ Гайка шестигранная самоконтрящаяся - Сталь метрическая Property Class 5 and 10 - Metric M5 x 0.8 Металлич.:27
- Вставка:99 [Insert]: Side_bar:4 ↔ Гайка шестигранная самоконтрящаяся - Сталь метрическая Property Class 5 and 10 - Metric M5 x 0.8 Металлич.:28
- Вставка:100 [Insert]: Side_bar:4 ↔ Гайка шестигранная самоконтрящаяся - Сталь метрическая Property Class 5 and 10 - Metric M5 x 0.8 Металлич.:29
- Вставка:101 [Insert]: Side_bar:2 ↔ Гайка шестигранная самоконтрящаяся - Сталь метрическая Property Class 5 and 10 - Metric M5 x 0.8 Металлич.:30
- Вставка:102 [Insert]: Side_bar:2 ↔ Гайка шестигранная самоконтрящаяся - Сталь метрическая Property Class 5 and 10 - Metric M5 x 0.8 Металлич.:31
- Вставка:103 [Insert]: Side_bar:2 ↔ Гайка шестигранная самоконтрящаяся - Сталь метрическая Property Class 5 and 10 - Metric M5 x 0.8 Металлич.:32
- Вставка:104 [Insert]: PCB_cover:1 ↔ Гайка шестигранная самоконтрящаяся - Сталь метрическая Property Class 5 and 10 - Metric M5 x 0.8 Металлич.:33
## Named parameters: sa_0 = 100000
note: some values were not read from the file. Shown as the stored number, unit unknown: "sa_0".
